# Autodesk Inventor assembly: FrameV2
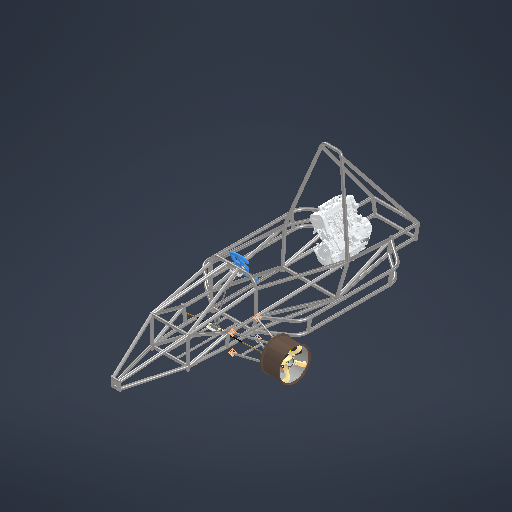
[picture p0: Inventor's stored thumbnail of the model, 512x512]
Saved by Autodesk Inventor 2026.2 (Build 302298010, 298A)
## iProperties
Created: 2026-06-05
Part Number: FrameV2
Document SubType Name: Assembly
Designer: tasle
_SolveAssemblyDoc: Frame Generator Solve Assembly
_Version: 15.0.0
Author: tasle
## Documents named in this file (11)
- C:\Users\tasle\Documents\PersonalProjects\FSAE\GOGO_FSAE_CAD\FrameV2.iam
- C:\Users\tasle\Documents\PersonalProjects\FSAE\GOGO_FSAE_CAD\PrelimFrame.ipt
- C:\Users\tasle\Documents\PersonalProjects\FSAE\GOGO_FSAE_CAD\FrameV2\Frame\Frame 1780692296746.iam
- C:\Users\tasle\Documents\PersonalProjects\FSAE\GOGO_FSAE_CAD\honda-cbr600-f4i-engine-1.snapshot.3\Honda CBR600 F4i\Honda CBR600 F4i\Honda CBR600 F4i.ipt
- C:\Users\tasle\Documents\PersonalProjects\FSAE\GOGO_FSAE_CAD\Suspension\Upright Assembly\Front Left Wheel Hub Assemby.iam
- C:\Users\tasle\Documents\PersonalProjects\FSAE\GOGO_FSAE_CAD\Suspension\Suspension Parts\Front Upper Arm\Front_Upper_Arm_Assembly.iam
- C:\Users\tasle\Documents\PersonalProjects\FSAE\GOGO_FSAE_CAD\Steering\SteeringAssy.iam
- C:\Users\tasle\Documents\PersonalProjects\FSAE\GOGO_FSAE_CAD\Steering\steeringmountplate.ipt
- C:\Users\tasle\Documents\PersonalProjects\FSAE\GOGO_FSAE_CAD\Steering\steeringbracket.ipt
- C:\Users\tasle\Documents\PersonalProjects\FSAE\GOGO_FSAE_CAD\Steering\rackmountplate.ipt
- C:\Users\tasle\Documents\PersonalProjects\FSAE\GOGO_FSAE_CAD\Steering\rackbracket.ipt
## Components (12 placed, 10 different names)
1. PrelimFrame:1 — Rotational:3
2. Frame 1780692296746:1 [sub-assembly] — Tangent:1, Tangent:2
3. Honda CBR600 F4i:1
4. Front Left Wheel Hub Assemby:1 [sub-assembly] — Rotational:1, Rotational:2
5. Front_Upper_Arm_Assembly:1 [sub-assembly] — Rotational:1
6. Front_Upper_Arm_Assembly:2 [sub-assembly] — Rotational:2
7. SteeringAssy:1 [sub-assembly] — Rigid:1, Mate:4
8. steeringmountplate:1 — Rotational:3, Mate:1, Mate:2, Mate:3
9. steeringbracket:1 — Mate:1, Mate:2, Mate:3, Rigid:1
10. rackmountplate:1 — Tangent:1, Tangent:2, Rigid:2, Rigid:3
11. rackbracket:1 — Rigid:3, Mate:4
12. rackbracket:2 — Rigid:2
## Relationships (12: Mate 4, RevoluteJoint 3, WeldJoint 3, Tangent 2)
- Rotational:1 [RevoluteJoint]: Front Left Wheel Hub Assemby:1 ↔ Front_Upper_Arm_Assembly:1
- Rotational:2 [RevoluteJoint]: Front Left Wheel Hub Assemby:1 ↔ Front_Upper_Arm_Assembly:2
- Rotational:3 [RevoluteJoint] (-20 mm): PrelimFrame:1 ↔ steeringmountplate:1
- Mate:1: steeringmountplate:1 ↔ steeringbracket:1
- Mate:2: steeringmountplate:1 ↔ steeringbracket:1
- Mate:3: steeringmountplate:1 ↔ steeringbracket:1
- Rigid:1 [WeldJoint]: SteeringAssy:1 ↔ steeringbracket:1
- Tangent:1: Frame 1780692296746:1 ↔ rackmountplate:1
- Tangent:2: Frame 1780692296746:1 ↔ rackmountplate:1
- Rigid:2 [WeldJoint]: rackmountplate:1 ↔ rackbracket:2
- Rigid:3 [WeldJoint]: rackmountplate:1 ↔ rackbracket:1
- Mate:4: SteeringAssy:1 ↔ rackbracket:1
